# Autodesk Inventor assembly: 24_0497_0001
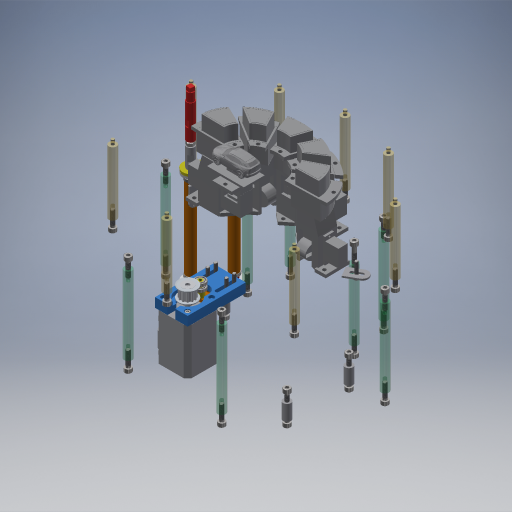
[picture p0: Inventor's stored thumbnail of the model, 512x512]
Saved by Autodesk Inventor 2024.3 (Build 283343000, 343)
## iProperties
Created: 2024-05-28
Part Number: 24_0497_0001
Document SubType Name: Assembly
Designer: Vogel
Author: Vogel
## Documents named in this file (37)
- D:\CAD\240497 - Kompass, Gehäuse\24_0497_0001.iam
- D:\CAD\240497 - Kompass, Gehäuse\24_0497_001.ipt
- D:\CAD\240497 - Kompass, Gehäuse\24_0497_002.ipt
- D:\CAD\240497 - Kompass, Gehäuse\24_0497_003.ipt
- D:\CAD\240497 - Kompass, Gehäuse\24_0497_004.ipt
- D:\CAD\240497 - Kompass, Gehäuse\24_0497_005.ipt
- D:\CAD\240497 - Kompass, Gehäuse\Motor ST4118D1804-A.ipt
- D:\CAD\240497 - Kompass, Gehäuse\24_0497_006.ipt
- D:\CAD\240497 - Kompass, Gehäuse\Alle_Schalter.ipt
- D:\CAD\240497 - Kompass, Gehäuse\abgerundete_buttons.ipt
- C:\Users\Vogel\Documents\Inventor\Content Center Files\R2024\de-DE\DIN BEARING(1)\DIN 625 SKF - SKF 618_6.ipt
- D:\CAD\240497 - Kompass, Gehäuse\Kaufteile\MAEDLER_16221200\16221200.ipt
- D:\CAD\240497 - Kompass, Gehäuse\24_0497_007.ipt
- D:\CAD\240497 - Kompass, Gehäuse\24_0497_008.ipt
- D:\CAD\240497 - Kompass, Gehäuse\24_0497_009.ipt
- D:\CAD\240497 - Kompass, Gehäuse\24_0497_0011.ipt
- D:\CAD\240497 - Kompass, Gehäuse\24_0497_0012.ipt
- D:\CAD\240497 - Kompass, Gehäuse\24_0497_0013.ipt
- D:\CAD\240497 - Kompass, Gehäuse\24_0497_0014.ipt
- D:\CAD\240497 - Kompass, Gehäuse\24_0497_0015.ipt
- D:\CAD\240497 - Kompass, Gehäuse\24_0497_0016.ipt
- D:\CAD\240497 - Kompass, Gehäuse\24_0497_0017.ipt
- C:\Users\Vogel\Documents\Inventor\Content Center Files\R2024\de-DE\DIN EN ISO 4032\DIN EN ISO 4032 - M5.ipt
- C:\Users\Vogel\Documents\Inventor\Content Center Files\R2024\de-DE\ISO 4762(1)\DIN EN ISO 4762 - M5 x 12.ipt
- C:\Users\Vogel\Documents\Inventor\Content Center Files\R2024\de-DE\ISO 4762(1)\DIN EN ISO 4762 - M5 x 20.ipt
- C:\Users\Vogel\Documents\Inventor\Content Center Files\R2024\de-DE\ISO 4762(1)\DIN EN ISO 4762 - M5 x 16.ipt
- C:\Users\Vogel\Documents\Inventor\Content Center Files\R2024\de-DE\ISO 4762(1)\DIN EN ISO 4762 - M3 x 16.ipt
- C:\Users\Vogel\Documents\Inventor\Content Center Files\R2024\de-DE\ISO 4762(1)\DIN EN ISO 4762 - M4 x 16.ipt
- C:\Users\Vogel\Documents\Inventor\Content Center Files\R2024\de-DE\ISO 10642(2)\ISO 10642  - M4  x  12.ipt
- C:\Users\Vogel\Documents\Inventor\Content Center Files\R2024\de-DE\ISO 2338(1)\DIN EN ISO 2338 - 3 h8 x 10.ipt
- D:\CAD\240497 - Kompass, Gehäuse\24_0497_0018.ipt
- D:\CAD\240497 - Kompass, Gehäuse\24_0497_0019.ipt
- D:\CAD\240497 - Kompass, Gehäuse\24_0497_0020.ipt
- C:\Users\Vogel\Documents\Inventor\Content Center Files\R2024\de-DE\ISO 4762(1)\DIN EN ISO 4762 - M5 x 30.ipt
- D:\CAD\240497 - Kompass, Gehäuse\Motor ST nema 23.ipt
- D:\CAD\240497 - Kompass, Gehäuse\24_0497_0021.ipt
- D:\CAD\240497 - Kompass, Gehäuse\24_0497_0022.ipt
## Components (104 placed, 36 different names)
1. 24_0497_001:1 — Passend:1, Fluchtend:1, Fluchtend:2, Einfügen:17, Einfügen:18, Einfügen:19, Einfügen:20, Einfügen:21, Einfügen:22, Einfügen:23, Einfügen:24, Passend:25, Fluchtend:22, Fluchtend:23, Passend:34, Passend:35
2. 24_0497_002:1 — Passend:1, Fluchtend:1, Fluchtend:2, Passend:2, Fluchtend:3, Fluchtend:4, Fluchtend:7, Fluchtend:8, Fluchtend:9, Fluchtend:16, Tangential:6, Fluchtend:18, Tangential:7
3. 24_0497_003:1 — Passend:2, Fluchtend:3, Fluchtend:4, Passend:3, Passend:4, Einfügen:33, Einfügen:34, Einfügen:35, Einfügen:36, Einfügen:47, Einfügen:48, Einfügen:49, Einfügen:50, Einfügen:51, Einfügen:52, Einfügen:53, Einfügen:54, Einfügen:55, Einfügen:56, Einfügen:79, Einfügen:80
4. 24_0497_004:1 — Einfügen:4, Einfügen:5, Fluchtend:19, Einfügen:9, Einfügen:11, Passend:6, Winkel:1, Fluchtend:20, Einfügen:13, Passend:7, Einfügen:39, Einfügen:41
5. 24_0497_004:2 — Einfügen:6, Einfügen:7, Fluchtend:16, Fluchtend:18, Fluchtend:19, Einfügen:8, Einfügen:10, Einfügen:15, Passend:9, Einfügen:38, Einfügen:40
6. Motor ST4118D1804-A:1 — Passend:3, Passend:4, Einfügen:12, Einfügen:14, Passend:8, Einfügen:83
7. 24_0497_006:1 — Fluchtend:7, Fluchtend:8, Fluchtend:9, Passend:5, Einfügen:27, Einfügen:28, Einfügen:29, Einfügen:30, Einfügen:31, Einfügen:32, Einfügen:57, Einfügen:58, Einfügen:59, Einfügen:60, Einfügen:61, Einfügen:62, Einfügen:63, Einfügen:64, Einfügen:65, Einfügen:66, Einfügen:67, Einfügen:68, Einfügen:69, Einfügen:70, Passend:15, Passend:17, Passend:19, Passend:21, Passend:26, Passend:27, Passend:28, Passend:29, Tangential:8, Tangential:9, Passend:30, Passend:32, Einfügen:77, Einfügen:78, Einfügen:81, Einfügen:82
8. Alle_Schalter:1 — Passend:5, Fluchtend:13, Fluchtend:14, Fluchtend:15
9. abgerundete_buttons:1 — Fluchtend:13, Fluchtend:14, Fluchtend:15
10. DIN 625 SKF SKF 618/6:1 — Einfügen:6, Tangential:6
11. DIN 625 SKF SKF 618/6:2 — Einfügen:4, Tangential:7
12. DIN 625 SKF SKF 618/6:3 — Einfügen:5
13. DIN 625 SKF SKF 618/6:4 — Einfügen:7
14. 24_0497_005:1 — Einfügen:8, Einfügen:9, Einfügen:16, Einfügen:25, Einfügen:42, Einfügen:71
15. 24_0497_005:2 — Einfügen:10, Einfügen:11, Einfügen:26, Passend:11, Einfügen:72, Einfügen:73
16. 16221200:1 — Einfügen:12
17. 24_0497_007:1 — Passend:6, Winkel:1, Fluchtend:20, Einfügen:13, Passend:7, Passend:23, Einfügen:76
18. 24_0497_007:2 — Einfügen:15, Passend:9, Passend:24, Einfügen:75
19. 24_0497_008:1 — Einfügen:14, Passend:8, Einfügen:74, Passend:16, Passend:18, Passend:20, Passend:22, Passend:36, Passend:37
20. 24_0497_009:1 — Einfügen:16, Passend:10
21. 24_0497_0011:1 — Einfügen:20
22. 24_0497_0011:2 — Einfügen:21
23. 24_0497_0011:3 — Einfügen:17
24. 24_0497_0011:4 — Einfügen:18
25. 24_0497_0011:5 — Einfügen:19
26. 24_0497_0011:6 — Einfügen:24
27. 24_0497_0011:7 — Einfügen:23
28. 24_0497_0011:8 — Einfügen:22
29. 24_0497_0012:1 — Einfügen:25, Passend:10
30. 24_0497_0012:2 — Einfügen:26, Passend:11
31. 24_0497_0013:1 — Einfügen:33
32. 24_0497_0013:2 — Einfügen:34, Einfügen:37
33. 24_0497_0013:3 — Einfügen:35
34. 24_0497_0013:4 — Einfügen:36, Passend:12
35. 24_0497_0014:1 — Einfügen:27
36. 24_0497_0014:2 — Einfügen:28
37. 24_0497_0014:3 — Einfügen:29
38. 24_0497_0014:4 — Einfügen:31
39. 24_0497_0014:5 — Einfügen:30
40. 24_0497_0014:6 — Einfügen:32
41. 24_0497_0015:1 — Einfügen:37, Passend:12, Einfügen:43, Einfügen:44, Einfügen:45, Einfügen:46
42. 24_0497_0016:1 — Einfügen:41
43. 24_0497_0016:2 — Einfügen:40
44. 24_0497_0016:3 — Einfügen:39
45. 24_0497_0016:4 — Einfügen:38
46. 24_0497_0017:1 — Einfügen:42, Passend:13, Passend:14
47. 24_0497_0018:1 — Passend:25, Fluchtend:21, Fluchtend:22, Fluchtend:23
48. 24_0497_0018:2 — Fluchtend:21, Passend:34, Passend:35
49. DIN EN ISO 4032 M5:1 — Passend:13, Passend:14
50. DIN EN ISO 4762 M5 x 12:1 — Einfügen:43
51. DIN EN ISO 4762 M5 x 12:2 — Einfügen:44
52. DIN EN ISO 4762 M5 x 12:3 — Einfügen:45
53. DIN EN ISO 4762 M5 x 12:4 — Einfügen:46
54. DIN EN ISO 4762 M5 x 20:1 — Einfügen:47
55. DIN EN ISO 4762 M5 x 20:2 — Einfügen:48
56. DIN EN ISO 4762 M5 x 20:3 — Einfügen:49
57. DIN EN ISO 4762 M5 x 20:4 — Einfügen:50
58. DIN EN ISO 4762 M5 x 20:5 — Einfügen:51
59. DIN EN ISO 4762 M5 x 20:6 — Einfügen:52
60. DIN EN ISO 4762 M5 x 20:7 — Einfügen:53
61. DIN EN ISO 4762 M5 x 20:8 — Einfügen:54
62. DIN EN ISO 4762 M5 x 20:9 — Einfügen:55
63. DIN EN ISO 4762 M5 x 20:10 — Einfügen:56
64. DIN EN ISO 4762 M5 x 20:11 — Einfügen:57
65. DIN EN ISO 4762 M5 x 20:12 — Einfügen:58
66. DIN EN ISO 4762 M5 x 20:13 — Einfügen:59
67. DIN EN ISO 4762 M5 x 20:14 — Einfügen:60
68. DIN EN ISO 4762 M5 x 20:15 — Einfügen:61
69. DIN EN ISO 4762 M5 x 20:16 — Einfügen:62
70. DIN EN ISO 4762 M5 x 20:17 — Einfügen:63
71. DIN EN ISO 4762 M5 x 20:18 — Einfügen:64
72. DIN EN ISO 4762 M5 x 20:19 — Einfügen:65
73. DIN EN ISO 4762 M5 x 20:20 — Einfügen:66
74. DIN EN ISO 4762 M5 x 20:21 — Einfügen:67
75. DIN EN ISO 4762 M5 x 20:22 — Einfügen:68
76. DIN EN ISO 4762 M5 x 20:23 — Einfügen:69
77. DIN EN ISO 4762 M5 x 20:24 — Einfügen:70
78. DIN EN ISO 4762 M5 x 16:1 — Einfügen:71
79. DIN EN ISO 4762 M5 x 16:2 — Einfügen:72
80. DIN EN ISO 4762 M5 x 16:3 — Einfügen:73
81. DIN EN ISO 4762 M3 x 16:1 — Einfügen:74
82. DIN EN ISO 4762 M4 x 16:1 — Passend:15, Passend:16
83. DIN EN ISO 4762 M4 x 16:3 — Passend:17, Passend:18
84. DIN EN ISO 4762 M4 x 16:4 — Passend:19, Passend:20
85. DIN EN ISO 4762 M4 x 16:5 — Passend:21, Passend:22
86. DIN EN ISO 10642 M4  x  12:1 — Passend:23
87. DIN EN ISO 10642 M4  x  12:2 — Passend:24
88. DIN EN ISO 2338 3 h8 x 10:1 — Einfügen:76
89. DIN EN ISO 2338 3 h8 x 10:2 — Einfügen:75
90. 24_0497_0019:1 — Passend:28, Passend:29, Tangential:8, Passend:33
91. 24_0497_0019:2 — Passend:26, Passend:27, Tangential:9, Passend:31
92. DIN EN ISO 4762 M4 x 16:6 — Passend:30, Passend:31
93. DIN EN ISO 4762 M4 x 16:7 — Passend:32, Passend:33
94. 24_0497_0020:1 — Einfügen:77
95. 24_0497_0020:2 — Einfügen:78
96. DIN EN ISO 4762 M5 x 20:25 — Einfügen:79
97. DIN EN ISO 4762 M5 x 20:26 — Einfügen:80
98. DIN EN ISO 4762 M5 x 30:1 — Einfügen:81
99. DIN EN ISO 4762 M5 x 30:2 — Einfügen:82
100. Motor ST nema 23:1 — Einfügen:83
101. 24_0497_0021:1 — Passend:36, Passend:37, Einfügen:84
102. 24_0497_0022:1 — Einfügen:84, Einfügen:85
103. DIN 625 SKF SKF 618/6:5 — Einfügen:85, Einfügen:86
104. DIN 625 SKF SKF 618/6:6 — Einfügen:86
## Relationships (142: Insert 83, Mate 37, Flush 17, Tangent 4, Angle 1)
- Passend:1 [Mate] (82 mm): 24_0497_001:1 ↔ 24_0497_002:1
- Fluchtend:1 [Flush]: 24_0497_001:1 ↔ 24_0497_002:1
- Fluchtend:2 [Flush]: 24_0497_001:1 ↔ 24_0497_002:1
- Passend:2 [Mate] (100 mm): 24_0497_002:1 ↔ 24_0497_003:1
- Fluchtend:3 [Flush]: 24_0497_002:1 ↔ 24_0497_003:1
- Fluchtend:4 [Flush]: 24_0497_002:1 ↔ 24_0497_003:1
- Passend:3 [Mate] (18 mm): 24_0497_003:1 ↔ Motor ST4118D1804-A:1
- Fluchtend:7 [Flush]: 24_0497_002:1 ↔ 24_0497_006:1
- Fluchtend:8 [Flush]: 24_0497_002:1 ↔ 24_0497_006:1
- Fluchtend:9 [Flush]: 24_0497_002:1 ↔ 24_0497_006:1
- Passend:4 [Mate]: 24_0497_003:1 ↔ Motor ST4118D1804-A:1
- Passend:5 [Mate]: 24_0497_006:1 ↔ Alle_Schalter:1
- Fluchtend:13 [Flush]: Alle_Schalter:1 ↔ abgerundete_buttons:1
- Fluchtend:14 [Flush]: Alle_Schalter:1 ↔ abgerundete_buttons:1
- Fluchtend:15 [Flush]: Alle_Schalter:1 ↔ abgerundete_buttons:1
- Einfügen:4 [Insert]: 24_0497_004:1 ↔ DIN 625 SKF SKF 618/6:2
- Einfügen:5 [Insert]: 24_0497_004:1 ↔ DIN 625 SKF SKF 618/6:3
- Einfügen:6 [Insert]: 24_0497_004:2 ↔ DIN 625 SKF SKF 618/6:1
- Einfügen:7 [Insert]: 24_0497_004:2 ↔ DIN 625 SKF SKF 618/6:4
- Fluchtend:16 [Flush]: 24_0497_002:1 ↔ 24_0497_004:2
- Tangential:6: 24_0497_002:1 ↔ DIN 625 SKF SKF 618/6:1
- Fluchtend:18 [Flush]: 24_0497_002:1 ↔ 24_0497_004:2
- Fluchtend:19 [Flush]: 24_0497_004:1 ↔ 24_0497_004:2
- Tangential:7: 24_0497_002:1 ↔ DIN 625 SKF SKF 618/6:2
- Einfügen:8 [Insert] (3 mm): 24_0497_004:2 ↔ 24_0497_005:1
- Einfügen:9 [Insert] (3 mm): 24_0497_004:1 ↔ 24_0497_005:1
- Einfügen:10 [Insert] (3 mm): 24_0497_004:2 ↔ 24_0497_005:2
- Einfügen:11 [Insert] (3 mm): 24_0497_004:1 ↔ 24_0497_005:2
- Einfügen:12 [Insert] (-2 mm): Motor ST4118D1804-A:1 ↔ 16221200:1
- Passend:6 [Mate]: 24_0497_004:1 ↔ 24_0497_007:1
- Winkel:1 [Angle] (0 deg): 24_0497_004:1 ↔ 24_0497_007:1
- Fluchtend:20 [Flush] (-3 mm): 24_0497_004:1 ↔ 24_0497_007:1
- Einfügen:13 [Insert]: 24_0497_004:1 ↔ 24_0497_007:1
- Passend:7 [Mate]: 24_0497_004:1 ↔ 24_0497_007:1
- Einfügen:14 [Insert]: Motor ST4118D1804-A:1 ↔ 24_0497_008:1
- Passend:8 [Mate]: Motor ST4118D1804-A:1 ↔ 24_0497_008:1
- Einfügen:15 [Insert]: 24_0497_004:2 ↔ 24_0497_007:2
- Passend:9 [Mate]: 24_0497_004:2 ↔ 24_0497_007:2
- Einfügen:16 [Insert] (31 mm): 24_0497_005:1 ↔ 24_0497_009:1
- Einfügen:17 [Insert]: 24_0497_001:1 ↔ 24_0497_0011:3
- Einfügen:18 [Insert]: 24_0497_001:1 ↔ 24_0497_0011:4
- Einfügen:19 [Insert]: 24_0497_001:1 ↔ 24_0497_0011:5
- Einfügen:20 [Insert]: 24_0497_001:1 ↔ 24_0497_0011:1
- Einfügen:21 [Insert]: 24_0497_001:1 ↔ 24_0497_0011:2
- Einfügen:22 [Insert]: 24_0497_001:1 ↔ 24_0497_0011:8
- Einfügen:23 [Insert]: 24_0497_001:1 ↔ 24_0497_0011:7
- Einfügen:24 [Insert]: 24_0497_001:1 ↔ 24_0497_0011:6
- Einfügen:25 [Insert]: 24_0497_005:1 ↔ 24_0497_0012:1
- Passend:10 [Mate]: 24_0497_009:1 ↔ 24_0497_0012:1
- Einfügen:26 [Insert]: 24_0497_005:2 ↔ 24_0497_0012:2
- Passend:11 [Mate]: 24_0497_005:2 ↔ 24_0497_0012:2
- Einfügen:27 [Insert]: 24_0497_006:1 ↔ 24_0497_0014:1
- Einfügen:28 [Insert]: 24_0497_006:1 ↔ 24_0497_0014:2
- Einfügen:29 [Insert]: 24_0497_006:1 ↔ 24_0497_0014:3
- Einfügen:30 [Insert]: 24_0497_006:1 ↔ 24_0497_0014:5
- Einfügen:31 [Insert]: 24_0497_006:1 ↔ 24_0497_0014:4
- Einfügen:32 [Insert]: 24_0497_006:1 ↔ 24_0497_0014:6
- Einfügen:33 [Insert]: 24_0497_003:1 ↔ 24_0497_0013:1
- Einfügen:34 [Insert]: 24_0497_003:1 ↔ 24_0497_0013:2
- Einfügen:35 [Insert]: 24_0497_003:1 ↔ 24_0497_0013:3
- Einfügen:36 [Insert]: 24_0497_003:1 ↔ 24_0497_0013:4
- Einfügen:37 [Insert]: 24_0497_0013:2 ↔ 24_0497_0015:1
- Passend:12 [Mate]: 24_0497_0013:4 ↔ 24_0497_0015:1
- Einfügen:38 [Insert]: 24_0497_004:2 ↔ 24_0497_0016:4
- Einfügen:39 [Insert]: 24_0497_004:1 ↔ 24_0497_0016:3
- Einfügen:40 [Insert]: 24_0497_004:2 ↔ 24_0497_0016:2
- Einfügen:41 [Insert]: 24_0497_004:1 ↔ 24_0497_0016:1
- Einfügen:42 [Insert]: 24_0497_005:1 ↔ 24_0497_0017:1
- Passend:13 [Mate]: 24_0497_0017:1 ↔ DIN EN ISO 4032 M5:1
- Passend:14 [Mate]: 24_0497_0017:1 ↔ DIN EN ISO 4032 M5:1
- Einfügen:43 [Insert]: 24_0497_0015:1 ↔ DIN EN ISO 4762 M5 x 12:1
- Einfügen:44 [Insert]: 24_0497_0015:1 ↔ DIN EN ISO 4762 M5 x 12:2
- Einfügen:45 [Insert]: 24_0497_0015:1 ↔ DIN EN ISO 4762 M5 x 12:3
- Einfügen:46 [Insert]: 24_0497_0015:1 ↔ DIN EN ISO 4762 M5 x 12:4
- Einfügen:47 [Insert]: 24_0497_003:1 ↔ DIN EN ISO 4762 M5 x 20:1
- Einfügen:48 [Insert]: 24_0497_003:1 ↔ DIN EN ISO 4762 M5 x 20:2
- Einfügen:49 [Insert]: 24_0497_003:1 ↔ DIN EN ISO 4762 M5 x 20:3
- Einfügen:50 [Insert]: 24_0497_003:1 ↔ DIN EN ISO 4762 M5 x 20:4
- Einfügen:51 [Insert]: 24_0497_003:1 ↔ DIN EN ISO 4762 M5 x 20:5
- Einfügen:52 [Insert]: 24_0497_003:1 ↔ DIN EN ISO 4762 M5 x 20:6
- Einfügen:53 [Insert]: 24_0497_003:1 ↔ DIN EN ISO 4762 M5 x 20:7
- Einfügen:54 [Insert]: 24_0497_003:1 ↔ DIN EN ISO 4762 M5 x 20:8
- Einfügen:55 [Insert]: 24_0497_003:1 ↔ DIN EN ISO 4762 M5 x 20:9
- Einfügen:56 [Insert]: 24_0497_003:1 ↔ DIN EN ISO 4762 M5 x 20:10
- Einfügen:57 [Insert]: 24_0497_006:1 ↔ DIN EN ISO 4762 M5 x 20:11
- Einfügen:58 [Insert]: 24_0497_006:1 ↔ DIN EN ISO 4762 M5 x 20:12
- Einfügen:59 [Insert]: 24_0497_006:1 ↔ DIN EN ISO 4762 M5 x 20:13
- Einfügen:60 [Insert]: 24_0497_006:1 ↔ DIN EN ISO 4762 M5 x 20:14
- Einfügen:61 [Insert]: 24_0497_006:1 ↔ DIN EN ISO 4762 M5 x 20:15
- Einfügen:62 [Insert]: 24_0497_006:1 ↔ DIN EN ISO 4762 M5 x 20:16
- Einfügen:63 [Insert]: 24_0497_006:1 ↔ DIN EN ISO 4762 M5 x 20:17
- Einfügen:64 [Insert]: 24_0497_006:1 ↔ DIN EN ISO 4762 M5 x 20:18
- Einfügen:65 [Insert]: 24_0497_006:1 ↔ DIN EN ISO 4762 M5 x 20:19
- Einfügen:66 [Insert]: 24_0497_006:1 ↔ DIN EN ISO 4762 M5 x 20:20
- Einfügen:67 [Insert]: 24_0497_006:1 ↔ DIN EN ISO 4762 M5 x 20:21
- Einfügen:68 [Insert]: 24_0497_006:1 ↔ DIN EN ISO 4762 M5 x 20:22
- Einfügen:69 [Insert]: 24_0497_006:1 ↔ DIN EN ISO 4762 M5 x 20:23
- Einfügen:70 [Insert]: 24_0497_006:1 ↔ DIN EN ISO 4762 M5 x 20:24
- Einfügen:71 [Insert]: 24_0497_005:1 ↔ DIN EN ISO 4762 M5 x 16:1
- Einfügen:72 [Insert]: 24_0497_005:2 ↔ DIN EN ISO 4762 M5 x 16:2
- Einfügen:73 [Insert]: 24_0497_005:2 ↔ DIN EN ISO 4762 M5 x 16:3
- Einfügen:74 [Insert]: 24_0497_008:1 ↔ DIN EN ISO 4762 M3 x 16:1
- Passend:15 [Mate]: 24_0497_006:1 ↔ DIN EN ISO 4762 M4 x 16:1
- Passend:16 [Mate]: 24_0497_008:1 ↔ DIN EN ISO 4762 M4 x 16:1
- Passend:17 [Mate]: 24_0497_006:1 ↔ DIN EN ISO 4762 M4 x 16:3
- Passend:18 [Mate]: 24_0497_008:1 ↔ DIN EN ISO 4762 M4 x 16:3
- Passend:19 [Mate]: 24_0497_006:1 ↔ DIN EN ISO 4762 M4 x 16:4
- Passend:20 [Mate]: 24_0497_008:1 ↔ DIN EN ISO 4762 M4 x 16:4
- Passend:21 [Mate]: 24_0497_006:1 ↔ DIN EN ISO 4762 M4 x 16:5
- Passend:22 [Mate]: 24_0497_008:1 ↔ DIN EN ISO 4762 M4 x 16:5
- Passend:23 [Mate]: 24_0497_007:1 ↔ DIN EN ISO 10642 M4  x  12:1
- Passend:24 [Mate]: 24_0497_007:2 ↔ DIN EN ISO 10642 M4  x  12:2
- Einfügen:75 [Insert]: 24_0497_007:2 ↔ DIN EN ISO 2338 3 h8 x 10:2
- Einfügen:76 [Insert]: 24_0497_007:1 ↔ DIN EN ISO 2338 3 h8 x 10:1
- Passend:25 [Mate]: 24_0497_001:1 ↔ 24_0497_0018:1
- Fluchtend:21 [Flush]: 24_0497_0018:1 ↔ 24_0497_0018:2
- Passend:26 [Mate]: 24_0497_006:1 ↔ 24_0497_0019:2
- Passend:27 [Mate]: 24_0497_006:1 ↔ 24_0497_0019:2
- Passend:28 [Mate]: 24_0497_006:1 ↔ 24_0497_0019:1
- Passend:29 [Mate]: 24_0497_006:1 ↔ 24_0497_0019:1
- Tangential:8: 24_0497_006:1 ↔ 24_0497_0019:1
- Tangential:9: 24_0497_006:1 ↔ 24_0497_0019:2
- Passend:30 [Mate]: 24_0497_006:1 ↔ DIN EN ISO 4762 M4 x 16:6
- Passend:31 [Mate]: 24_0497_0019:2 ↔ DIN EN ISO 4762 M4 x 16:6
- Passend:32 [Mate]: 24_0497_006:1 ↔ DIN EN ISO 4762 M4 x 16:7
- Passend:33 [Mate]: 24_0497_0019:1 ↔ DIN EN ISO 4762 M4 x 16:7
- Fluchtend:22 [Flush]: 24_0497_001:1 ↔ 24_0497_0018:1
- Fluchtend:23 [Flush]: 24_0497_001:1 ↔ 24_0497_0018:1
- Passend:34 [Mate]: 24_0497_001:1 ↔ 24_0497_0018:2
- Passend:35 [Mate]: 24_0497_001:1 ↔ 24_0497_0018:2
- Einfügen:77 [Insert]: 24_0497_006:1 ↔ 24_0497_0020:1
- Einfügen:78 [Insert]: 24_0497_006:1 ↔ 24_0497_0020:2
- Einfügen:79 [Insert]: 24_0497_003:1 ↔ DIN EN ISO 4762 M5 x 20:25
- Einfügen:80 [Insert]: 24_0497_003:1 ↔ DIN EN ISO 4762 M5 x 20:26
- Einfügen:81 [Insert]: 24_0497_006:1 ↔ DIN EN ISO 4762 M5 x 30:1
- Einfügen:82 [Insert]: 24_0497_006:1 ↔ DIN EN ISO 4762 M5 x 30:2
- Einfügen:83 [Insert]: Motor ST4118D1804-A:1 ↔ Motor ST nema 23:1
- Passend:36 [Mate]: 24_0497_008:1 ↔ 24_0497_0021:1
- Passend:37 [Mate]: 24_0497_008:1 ↔ 24_0497_0021:1
- Einfügen:84 [Insert]: 24_0497_0021:1 ↔ 24_0497_0022:1
- Einfügen:85 [Insert]: 24_0497_0022:1 ↔ DIN 625 SKF SKF 618/6:5
- Einfügen:86 [Insert] (3 mm): DIN 625 SKF SKF 618/6:5 ↔ DIN 625 SKF SKF 618/6:6
